# Autodesk Inventor assembly: Assembly1 vidalı artı parça
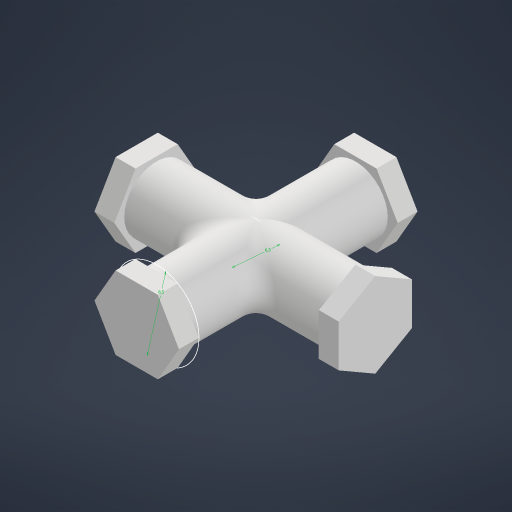
[picture p0: Inventor's stored thumbnail of the model, 512x512]
Saved by Autodesk Inventor 2023 (Build 270158030, 158C)
## iProperties
Created: 2023-03-11
Part Number: Assembly1 vidalı artı parça
Document SubType Name: Assembly
Designer: Monster
Author: Monster
## Documents named in this file (3)
- C:\Users\Monster\Desktop\Ders\UKA\shaft toplam\shaft imalat vida\Assembly1 vidalı artı parça.iam
- C:\Users\Monster\Desktop\Ders\UKA\shaft toplam\shaft imalat vida\shaft 4 kol.ipt
- C:\Users\Monster\Desktop\Ders\UKA\shaft toplam\shaft imalat vida\vida.ipt
## Components (5 placed, 2 different names)
1. shaft 4 kol:1 — Mate:1, Mate:2, Mate:3, Mate:4, Mate:5, Mate:6, Mate:7, Mate:8
2. vida:1 — Mate:2, Mate:5
3. vida:2 — Mate:1, Mate:7
4. vida:3 — Mate:4, Mate:8
5. vida:4 — Mate:3, Mate:6
## Relationships (8: Mate 8)
- Mate:1: shaft 4 kol:1 ↔ vida:2
- Mate:2: shaft 4 kol:1 ↔ vida:1
- Mate:3: shaft 4 kol:1 ↔ vida:4
- Mate:4: shaft 4 kol:1 ↔ vida:3
- Mate:5: shaft 4 kol:1 ↔ vida:1
- Mate:6: shaft 4 kol:1 ↔ vida:4
- Mate:7: shaft 4 kol:1 ↔ vida:2
- Mate:8: shaft 4 kol:1 ↔ vida:3
